# Autodesk Inventor assembly: Shadow_Game
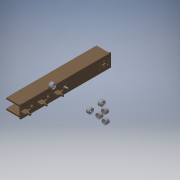
[picture p0: Inventor's stored thumbnail of the model, 180x180]
Saved by Autodesk Inventor 2016 (Build 200138000, 138)
## iProperties
Created: 2016-01-06
Part Number: Shadow_Game
Document SubType Name: Assembly
Designer: m2memari
Author: m2memari
## Documents named in this file (4)
- C:\MoDonGD\Jane\Series_2\Shadow_Game.iam
- C:\MoDonGD\Jane\Series_2\Motor_Bar.iam
- C:\MoDonGD\Jane\Series_2\SPG30_Motor.ipt
- C:\MoDonGD\Jane\Series_2\Bearing.ipt
## Components (8 placed, 3 different names)
1. Motor_Bar:1 [sub-assembly] — Insert:1, Tangent:1
2. SPG30_Motor:1 — Insert:1, Tangent:1
3. Bearing:1
4. Bearing:2
5. Bearing:3
6. Bearing:4
7. Bearing:5
8. Bearing:6
## Relationships (2: Insert 1, Tangent 1)
- Insert:1: Motor_Bar:1 ↔ SPG30_Motor:1
- Tangent:1: Motor_Bar:1 ↔ SPG30_Motor:1
